# Autodesk Inventor assembly: Sneak100_Zeta
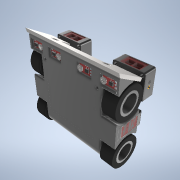
[picture p0: Inventor's stored thumbnail of the model, 180x180]
Saved by Autodesk Inventor 2021 (Build 250183000, 183)
## iProperties
Created: 2021-05-13
Part Number: Sneak100_Zeta
Document SubType Name: Assembly
Designer: ermoz
Author: ermoz
## Documents named in this file (15)
- D:\Moje Wyczyny\My_Poor_Projects\Sneak100_MiniSumo\minisumo-sneak100\mechanics\Sneak100_Zeta.iam
- D:\Moje Wyczyny\My_Poor_Projects\Sneak100_MiniSumo\minisumo-sneak100\mechanics\PreMadeParts\Pololu_MotorEncoderModule.iam
- D:\Moje Wyczyny\My_Poor_Projects\Sneak100_MiniSumo\minisumo-sneak100\mechanics\PreMadeParts\LiPO_2S_58x32x10.ipt
- D:\Moje Wyczyny\My_Poor_Projects\Sneak100_MiniSumo\minisumo-sneak100\mechanics\PreMadeParts\Solarbotics_RW2i.ipt
- D:\Moje Wyczyny\My_Poor_Projects\Sneak100_MiniSumo\minisumo-sneak100\mechanics\MechanicalElements\HullBottom.ipt
- D:\Moje Wyczyny\My_Poor_Projects\Sneak100_MiniSumo\minisumo-sneak100\mechanics\MechanicalElements\BatteryPlate.ipt
- D:\Moje Wyczyny\My_Poor_Projects\Sneak100_MiniSumo\minisumo-sneak100\mechanics\PreMadeParts\QTR1A.iam
- D:\Moje Wyczyny\My_Poor_Projects\Sneak100_MiniSumo\minisumo-sneak100\mechanics\PreMadeParts\M3_Short_Bolt.ipt
- D:\Moje Wyczyny\My_Poor_Projects\Sneak100_MiniSumo\minisumo-sneak100\mechanics\ModyfiedParts\HM_Knife_cut.ipt
- D:\Moje Wyczyny\My_Poor_Projects\Sneak100_MiniSumo\minisumo-sneak100\mechanics\PreMadeParts\3M_Nut.ipt
- D:\Moje Wyczyny\My_Poor_Projects\Sneak100_MiniSumo\minisumo-sneak100\mechanics\MechanicalElements\HullMid.ipt
- D:\Moje Wyczyny\My_Poor_Projects\Sneak100_MiniSumo\minisumo-sneak100\mechanics\MirroredParts\HullMid_MIR.ipt
- D:\Moje Wyczyny\My_Poor_Projects\Sneak100_MiniSumo\minisumo-sneak100\mechanics\MechanicalElements\HullTop.ipt
- D:\Moje Wyczyny\My_Poor_Projects\Sneak100_MiniSumo\minisumo-sneak100\mechanics\ElectricElements\MainModule.iam
- D:\Moje Wyczyny\My_Poor_Projects\Sneak100_MiniSumo\minisumo-sneak100\mechanics\PreMadeParts\20NK_3-50CM.ipt
## Components (32 placed, 14 different names)
1. Pololu_MotorEncoderModule:1 [sub-assembly] — Mate:1, Flush:1, Flush:3, Flush:5, Angle:1, Mate:6, Mate:7, Symmetry:1
2. Pololu_MotorEncoderModule:2 [sub-assembly] — Mate:2, Flush:2, Flush:3, Flush:5, Angle:2, Mate:6, Mate:9, Mate:11, Mate:15, Mate:16
3. Pololu_MotorEncoderModule:3 [sub-assembly] — Mate:1, Flush:1, Flush:4, Mate:8, Symmetry:1
4. Pololu_MotorEncoderModule:4 [sub-assembly] — Mate:2, Flush:2, Flush:4, Mate:10, Mate:11
5. LiPO_2S_58x32x10:1 — Mate:17, Mate:18, Mate:21
6. Solarbotics_RW2i:1 — Mate:3, Tangent:1, Mate:7, Flush:8, Symmetry:2
7. Solarbotics_RW2i:2 — Tangent:2, Mate:9, Flush:8, Flush:11
8. Solarbotics_RW2i:3 — Mate:3, Mate:8, Flush:7, Symmetry:2, Flush:22
9. Solarbotics_RW2i:4 — Mate:10, Flush:7
10. HullBottom:1 — Flush:11, Mate:15, Mate:16, Mate:17, Mate:18, Mate:19, Mate:20, Flush:18, Mate:26, Mate:27, Mate:28, Mate:29, Flush:25, Mate:38, Flush:26, Mate:39, Mate:41, Flush:28, Flush:29, Flush:31, Flush:34
11. BatteryPlate:1 — Mate:19, Mate:20, Mate:21, Flush:25
12. QTR1A:1 [sub-assembly] — Symmetry:4, Flush:14, Flush:17, Flush:18, Mate:22, Mate:27
13. QTR1A:2 [sub-assembly] — Symmetry:3, Flush:13, Flush:14, Flush:16, Flush:17, Mate:23, Mate:26, Mate:28
14. QTR1A:3 [sub-assembly] — Symmetry:3, Flush:12, Flush:13, Flush:15, Flush:16, Mate:24
15. QTR1A:4 [sub-assembly] — Symmetry:4, Flush:12, Flush:15, Mate:25
16. M3_Short_Bolt:1 — Mate:22, Flush:21
17. M3_Short_Bolt:2 — Mate:23, Flush:20, Flush:21
18. M3_Short_Bolt:3 — Mate:24, Flush:19, Flush:20
19. M3_Short_Bolt:4 — Mate:25, Flush:19
20. M3_Short_Bolt:5 — Symmetry:5, Flush:23, Mate:31, Mate:37
21. M3_Short_Bolt:6 — Symmetry:5, Flush:24, Mate:36
22. HM_Knife_cut:1 — Mate:29, Flush:22, Mate:30, Flush:23, Mate:31, Flush:24
23. 3M_Nut:5 — Mate:37
24. 3M_Nut:6 — Mate:36
25. HullMid:1 — Mate:38, Flush:26, Mate:39, Mate:44, Mate:45, Flush:30, Mate:46
26. HullMid_MIR:1 — Mate:41, Flush:28, Flush:29, Mate:43
27. HullTop:1 — Flush:30, Flush:31, Mate:46
28. MainModule:1 [sub-assembly] — Mate:43, Mate:44, Mate:45
29. 20NK_3-50CM:1 — Flush:32, Mate:47, Flush:33
30. 20NK_3-50CM:2 — Flush:32, Mate:47, Flush:33
31. 20NK_3-50CM:3 — Flush:34, Mate:48, Flush:35, Flush:36
32. 20NK_3-50CM:4 — Mate:48, Flush:35, Flush:36
## Relationships (78: Mate 37, Flush 32, Symmetry 5, Angle 2, Tangent 2)
- Mate:1: Pololu_MotorEncoderModule:1 ↔ Pololu_MotorEncoderModule:3
- Flush:1: Pololu_MotorEncoderModule:1 ↔ Pololu_MotorEncoderModule:3
- Mate:2: Pololu_MotorEncoderModule:2 ↔ Pololu_MotorEncoderModule:4
- Flush:2: Pololu_MotorEncoderModule:2 ↔ Pololu_MotorEncoderModule:4
- Flush:3: Pololu_MotorEncoderModule:1 ↔ Pololu_MotorEncoderModule:2
- Flush:4: Pololu_MotorEncoderModule:3 ↔ Pololu_MotorEncoderModule:4
- Flush:5: Pololu_MotorEncoderModule:1 ↔ Pololu_MotorEncoderModule:2
- Mate:3 (-98 mm): Solarbotics_RW2i:1 ↔ Solarbotics_RW2i:3
- Angle:1 (0 deg): Pololu_MotorEncoderModule:1
- Tangent:1: Solarbotics_RW2i:1
- Angle:2 (0 deg): Pololu_MotorEncoderModule:2
- Tangent:2: Solarbotics_RW2i:2
- Mate:6 (50 mm): Pololu_MotorEncoderModule:1 ↔ Pololu_MotorEncoderModule:2
- Mate:7: Pololu_MotorEncoderModule:1 ↔ Solarbotics_RW2i:1
- Mate:8: Pololu_MotorEncoderModule:3 ↔ Solarbotics_RW2i:3
- Mate:9: Pololu_MotorEncoderModule:2 ↔ Solarbotics_RW2i:2
- Mate:10: Pololu_MotorEncoderModule:4 ↔ Solarbotics_RW2i:4
- Flush:7: Solarbotics_RW2i:3 ↔ Solarbotics_RW2i:4
- Flush:8: Solarbotics_RW2i:1 ↔ Solarbotics_RW2i:2
- Mate:11 (-68 mm): Pololu_MotorEncoderModule:2 ↔ Pololu_MotorEncoderModule:4
- Symmetry:1: Pololu_MotorEncoderModule:1 ↔ Pololu_MotorEncoderModule:3
- Symmetry:2: Solarbotics_RW2i:1 ↔ Solarbotics_RW2i:3
- Flush:11: Solarbotics_RW2i:2 ↔ HullBottom:1
- Mate:15: Pololu_MotorEncoderModule:2 ↔ HullBottom:1
- Mate:16: Pololu_MotorEncoderModule:2 ↔ HullBottom:1
- Mate:17: LiPO_2S_58x32x10:1 ↔ HullBottom:1
- Mate:18 (1 mm): LiPO_2S_58x32x10:1 ↔ HullBottom:1
- Mate:19: HullBottom:1 ↔ BatteryPlate:1
- Mate:20: HullBottom:1 ↔ BatteryPlate:1
- Mate:21: LiPO_2S_58x32x10:1 ↔ BatteryPlate:1
- Symmetry:3: QTR1A:2 ↔ QTR1A:3
- Symmetry:4: QTR1A:1 ↔ QTR1A:4
- Flush:12: QTR1A:3 ↔ QTR1A:4
- Flush:13: QTR1A:2 ↔ QTR1A:3
- Flush:14: QTR1A:1 ↔ QTR1A:2
- Flush:15: QTR1A:3 ↔ QTR1A:4
- Flush:16: QTR1A:2 ↔ QTR1A:3
- Flush:17: QTR1A:1 ↔ QTR1A:2
- Flush:18: HullBottom:1 ↔ QTR1A:1
- Mate:22: QTR1A:1 ↔ M3_Short_Bolt:1
- Mate:23: QTR1A:2 ↔ M3_Short_Bolt:2
- Mate:24: QTR1A:3 ↔ M3_Short_Bolt:3
- Mate:25: QTR1A:4 ↔ M3_Short_Bolt:4
- Mate:26: HullBottom:1 ↔ QTR1A:2
- Mate:27: HullBottom:1 ↔ QTR1A:1
- Mate:28: HullBottom:1 ↔ QTR1A:2
- Flush:19: M3_Short_Bolt:3 ↔ M3_Short_Bolt:4
- Flush:20: M3_Short_Bolt:2 ↔ M3_Short_Bolt:3
- Flush:21: M3_Short_Bolt:1 ↔ M3_Short_Bolt:2
- Symmetry:5: M3_Short_Bolt:5 ↔ M3_Short_Bolt:6
- Mate:29: HullBottom:1 ↔ HM_Knife_cut:1
- Flush:22 (-1 mm): Solarbotics_RW2i:3 ↔ HM_Knife_cut:1
- Mate:30: HM_Knife_cut:1
- Flush:23: M3_Short_Bolt:5 ↔ HM_Knife_cut:1
- Mate:31: M3_Short_Bolt:5 ↔ HM_Knife_cut:1
- Flush:24: M3_Short_Bolt:6 ↔ HM_Knife_cut:1
- Flush:25: HullBottom:1 ↔ BatteryPlate:1
- Mate:36: M3_Short_Bolt:6 ↔ 3M_Nut:6
- Mate:37: M3_Short_Bolt:5 ↔ 3M_Nut:5
- Mate:38: HullBottom:1 ↔ HullMid:1
- Flush:26: HullBottom:1 ↔ HullMid:1
- Mate:39: HullBottom:1 ↔ HullMid:1
- Mate:41: HullBottom:1 ↔ HullMid_MIR:1
- Flush:28: HullBottom:1 ↔ HullMid_MIR:1
- Flush:29: HullBottom:1 ↔ HullMid_MIR:1
- Mate:43: HullMid_MIR:1 ↔ MainModule:1
- Mate:44: HullMid:1 ↔ MainModule:1
- Mate:45: HullMid:1 ↔ MainModule:1
- Flush:30: HullMid:1 ↔ HullTop:1
- Flush:31: HullBottom:1 ↔ HullTop:1
- Mate:46: HullMid:1 ↔ HullTop:1
- Flush:32: 20NK_3-50CM:1 ↔ 20NK_3-50CM:2
- Mate:47 (-98 mm): 20NK_3-50CM:1 ↔ 20NK_3-50CM:2
- Flush:33: 20NK_3-50CM:1 ↔ 20NK_3-50CM:2
- Flush:34: HullBottom:1 ↔ 20NK_3-50CM:3
- Mate:48 (-98 mm): 20NK_3-50CM:3 ↔ 20NK_3-50CM:4
- Flush:35: 20NK_3-50CM:3 ↔ 20NK_3-50CM:4
- Flush:36: 20NK_3-50CM:3 ↔ 20NK_3-50CM:4
